# Autodesk Inventor assembly: Locked CubeSat Assembly Frame
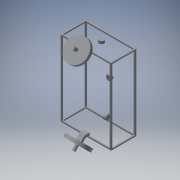
[picture p0: Inventor's stored thumbnail of the model, 180x180]
Saved by Autodesk Inventor 2016 (Build 200138000, 138)
## iProperties
Created: 2015-12-21
Part Number: Locked CubeSat Assembly Frame
Document SubType Name: Assembly
Designer: jonathan
Author: jonathan
## Documents named in this file (5)
- C:\Users\jshum\Dropbox\Satellite\CAD\Locked CubeSat Assembly Frame.iam
- C:\Users\jshum\Dropbox\Satellite\CAD\CubeSat Frame.ipt
- C:\Users\jshum\Dropbox\Satellite\CAD\Motor Assembly.iam
- C:\Users\jshum\Dropbox\Satellite\CAD\Orthogonal Bracket.ipt
- C:\Users\jshum\Dropbox\Satellite\CAD\Flywheel Bracket.ipt
## Components (8 placed, 4 different names)
1. CubeSat Frame:1 — Mate:4, Flush:3, Mate:6, Flush:4, Flush:5, Flush:6, Flush:7
2. Motor Assembly:1 [sub-assembly] — Mate:5, Rigid:1
3. Motor Assembly:2 [sub-assembly] — Rigid:2
4. Orthogonal Bracket:1 — Mate:4, Flush:3, Mate:5, Rigid:1
5. Orthogonal Bracket:2 — Mate:6, Flush:4, Rigid:2
6. Flywheel Bracket:1 — Flush:6
7. Flywheel Bracket:2 — Flush:5
8. Flywheel Bracket:3 — Flush:7
## Relationships (10: Flush 5, Mate 3, WeldJoint 2)
- Mate:4: CubeSat Frame:1 ↔ Orthogonal Bracket:1
- Flush:3: CubeSat Frame:1 ↔ Orthogonal Bracket:1
- Mate:5: Motor Assembly:1 ↔ Orthogonal Bracket:1
- Rigid:1 [WeldJoint]: Motor Assembly:1 ↔ Orthogonal Bracket:1
- Mate:6: CubeSat Frame:1 ↔ Orthogonal Bracket:2
- Flush:4: CubeSat Frame:1 ↔ Orthogonal Bracket:2
- Rigid:2 [WeldJoint]: Motor Assembly:2 ↔ Orthogonal Bracket:2
- Flush:5: CubeSat Frame:1 ↔ Flywheel Bracket:2
- Flush:6: CubeSat Frame:1 ↔ Flywheel Bracket:1
- Flush:7 (76.2 mm): CubeSat Frame:1 ↔ Flywheel Bracket:3
